# Autodesk Inventor assembly: PrinterMini
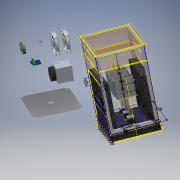
[picture p0: Inventor's stored thumbnail of the model, 180x180]
Saved by Autodesk Inventor 2016 (Build 200138000, 138)
## iProperties
Created: 2015-08-01
Part Number: PrinterMini
Document SubType Name: Assembly
Designer: myhome
Author: myhome
## Documents named in this file (15)
- C:\Users\myhome\Documents\Inventor\Printer\PrinterMini.iam
- C:\Users\myhome\Documents\Inventor\Printer\EpoxyGraniteBase\BaseMini.iam
- C:\Users\myhome\Documents\Inventor\Printer\FrameExtruded\FrameMini.iam
- C:\Users\myhome\Documents\Inventor\Printer\PistonFrame\PistonFeederFrameMini.iam
- C:\Users\myhome\Documents\Inventor\Printer\PistonFrame\PistonWorkFrameMini.iam
- C:\Users\myhome\Documents\Inventor\Printer\Nema17Motor\Nema17Stepper.iam
- C:\Users\myhome\Documents\Inventor\Printer\LinearActuator\LinearActuatorMini.iam
- C:\Users\myhome\Documents\Inventor\Printer\PistonHead\PistonFeederHeadMini.iam
- C:\Users\myhome\Documents\Inventor\Printer\FrameSheetMetal\FrameSheetLaserViewportMini.ipt
- C:\Users\myhome\Documents\Inventor\Printer\PistonHead\PistonWorkHeadMini.iam
- C:\Users\myhome\Documents\Inventor\Printer\SilverstoneFan\SilverstoneFQ121.iam
- C:\Users\myhome\Documents\Inventor\Printer\RaspberryPiCamera\RaspberryPiCamera.ipt
- C:\Users\myhome\Documents\Inventor\Printer\RaspberryPi2\RaspberryPi2.iam
- C:\Users\myhome\Documents\Inventor\Printer\GShield\GShield.iam
- C:\Users\myhome\Documents\Inventor\Printer\ScanCube\WarpCube.iam
## Components (21 placed, 14 different names)
1. BaseMini:1 [sub-assembly] — Rigid:1, Rigid:5, Rigid:10, Rigid:12
2. FrameMini:1 [sub-assembly] — Rigid:1
3. PistonFrameMini:1 [sub-assembly] — Mate:1
4. PistonWorkFrameMini:1 [sub-assembly] — Rigid:9
5. Nema17Stepper:1 [sub-assembly] — Rigid:5, Rotational:1
6. LinearActuatorMini:1 [sub-assembly] — Rigid:7, Rotational:2, Mate:1
7. LinearActuatorMini:3 [sub-assembly] — Rotational:1, Rigid:8, Rigid:9
8. PistonFeederHeadMini:3 [sub-assembly] — Rigid:7
9. FrameSheetLaserViewportMini:1
10. PistonWorkHeadMini:1 [sub-assembly] — Rigid:8
11. Nema17Stepper:2 [sub-assembly] — Rotational:2, Rigid:10
12. SilverstoneFQ121:2 [sub-assembly]
13. SilverstoneFQ121:3 [sub-assembly]
14. RaspberryPiCamera:1
15. RaspberryPi2:1 [sub-assembly]
16. GShield:1 [sub-assembly]
17. PistonFrameMini:3 [sub-assembly] — Mate:2
18. WarpCube:1 [sub-assembly]
19. PistonFeederHeadMini:4 [sub-assembly] — Rigid:11
20. LinearActuatorMini:8 [sub-assembly] — Rotational:3, Rigid:11, Mate:2
21. Nema17Stepper:4 [sub-assembly] — Rotational:3, Rigid:12
## Relationships (13: WeldJoint 8, RevoluteJoint 3, Mate 2)
- Rigid:1 [WeldJoint]: BaseMini:1 ↔ FrameMini:1
- Rigid:5 [WeldJoint]: BaseMini:1 ↔ Nema17Stepper:1
- Rotational:1 [RevoluteJoint]: Nema17Stepper:1 ↔ LinearActuatorMini:3
- Rigid:7 [WeldJoint]: LinearActuatorMini:1 ↔ PistonFeederHeadMini:3
- Rigid:8 [WeldJoint]: LinearActuatorMini:3 ↔ PistonWorkHeadMini:1
- Rigid:9 [WeldJoint]: PistonWorkFrameMini:1 ↔ LinearActuatorMini:3
- Rotational:2 [RevoluteJoint]: LinearActuatorMini:1 ↔ Nema17Stepper:2
- Mate:1: PistonFrameMini:1 ↔ LinearActuatorMini:1
- Rigid:10 [WeldJoint]: BaseMini:1 ↔ Nema17Stepper:2
- Rotational:3 [RevoluteJoint]: LinearActuatorMini:8 ↔ Nema17Stepper:4
- Rigid:11 [WeldJoint]: PistonFeederHeadMini:4 ↔ LinearActuatorMini:8
- Mate:2: PistonFrameMini:3 ↔ LinearActuatorMini:8
- Rigid:12 [WeldJoint]: BaseMini:1 ↔ Nema17Stepper:4
